# Autodesk Inventor assembly: legs_asm_alt
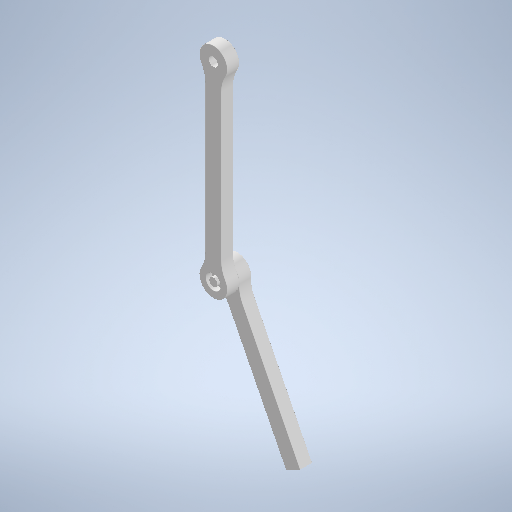
[picture p0: Inventor's stored thumbnail of the model, 512x512]
Saved by Autodesk Inventor 2025.1 (Build 291241000, 241)
## iProperties
Created: 2024-11-08
Part Number: legs_asm_alt
Document SubType Name: Assembly
Designer: ZOMBULLI
Author: ZOMBULLI
## Documents named in this file (4)
- C:\Users\xingj\Downloads\CAD\Stewart Platform_new\legs_asm_alt.iam
- C:\Users\xingj\Downloads\CAD\Stewart Platform_new\alternativeJoint - Kopie.ipt
- C:\Users\xingj\Downloads\CAD\Stewart Platform_new\alternativeJoint2 - Kopie.ipt
- C:\Users\xingj\Downloads\Part1.ipt
## Components (3 placed, 3 different names)
1. alternativeJoint - Kopie:1 — Mate:1, Mate:2, Angle:1, Mate:4, Mate:6, Mate:7, Mate:9
2. alternativeJoint2 - Kopie:1 — Mate:1, Mate:2, Angle:1, Flush:1, Mate:5, Mate:7, Mate:8, Flush:2
3. Part1:1 — Flush:1, Mate:4, Mate:5, Mate:6, Mate:8, Flush:2, Mate:9
## Relationships (11: Mate 8, Flush 2, Angle 1)
- Mate:1 (0.2 mm): alternativeJoint - Kopie:1 ↔ alternativeJoint2 - Kopie:1
- Mate:2: alternativeJoint - Kopie:1 ↔ alternativeJoint2 - Kopie:1
- Angle:1 (90 deg): alternativeJoint - Kopie:1 ↔ alternativeJoint2 - Kopie:1
- Flush:1: alternativeJoint2 - Kopie:1 ↔ Part1:1
- Mate:4: alternativeJoint - Kopie:1 ↔ Part1:1
- Mate:5: alternativeJoint2 - Kopie:1 ↔ Part1:1
- Mate:6: alternativeJoint - Kopie:1 ↔ Part1:1
- Mate:7: alternativeJoint - Kopie:1 ↔ alternativeJoint2 - Kopie:1
- Mate:8: alternativeJoint2 - Kopie:1 ↔ Part1:1
- Flush:2: alternativeJoint2 - Kopie:1 ↔ Part1:1
- Mate:9: alternativeJoint - Kopie:1 ↔ Part1:1
